# Autodesk Inventor assembly: MotorEncoderAssembly_MIR
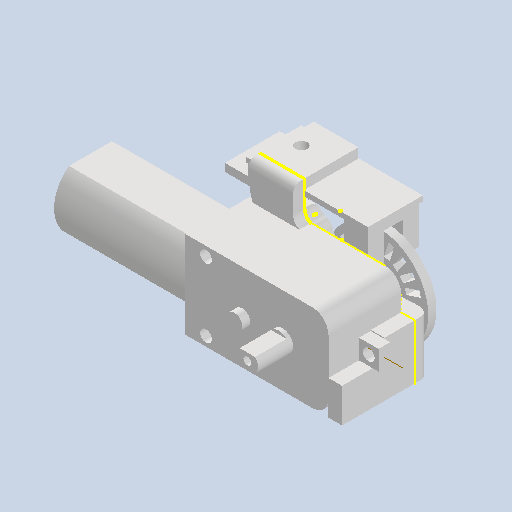
[picture p0: Inventor's stored thumbnail of the model, 512x512]
Saved by Autodesk Inventor 2022 (Build 260153070, 153G)
## iProperties
Created: 2021-11-27
Part Number: MotorEncoderAssembly_MIR
Document SubType Name: Assembly
Designer: a laptop
Author: a laptop
## Documents named in this file (8)
- C:\Users\a laptop\Desktop\SumoBot\sumobotENCODER\MotorEncoderAssembly_MIR.iam
- C:\Users\a laptop\Desktop\SumoBot\sumobotENCODER\REF_PART\LM393 encoder_MIR.ipt
- C:\Users\a laptop\Desktop\SumoBot\sumobotENCODER\REF_PART\TT encoder disk_MIR.ipt
- C:\Users\a laptop\Desktop\SumoBot\sumobotENCODER\REF_PART\TT motor output_MIR.ipt
- C:\Users\a laptop\Desktop\SumoBot\sumobotENCODER\MotorEncoderBracket_MIR.ipt
- C:\Users\a laptop\Desktop\SumoBot\sumobotENCODER\REF_PART\TTencoderspacer_MIR.ipt
- C:\Users\a laptop\Desktop\SumoBot\sumobotENCODER\REF_PART\TTencodercap_MIR.ipt
- C:\Users\a laptop\Desktop\SumoBot\sumobotENCODER\REF_PART\TTmotor_MIR.ipt
## Components (7 placed, 7 different names)
1. LM393 encoder_MIR:1 — Tangent:1, Mate:3, Angle:3, Angle:2, Mate:8
2. TT encoder disk_MIR:1 — Tangent:1, Mate:3, Mate:2, Flush:1, Angle:1, Mate:1
3. TT motor output_MIR:1 — Angle:3, Angle:2, Mate:2, Flush:1, Angle:1, Mate:1, Mate:4, Mate:5, Flush:2, Flush:3, Flush:4, Mate:11, Mate:10
4. MotorEncoderBracket_MIR:1 — Flush:2
5. TTencoderspacer_MIR:1 — Flush:3
6. TTencodercap_MIR:1 — Flush:4
7. TTmotor_MIR:1 — Mate:11, Mate:10
## Relationships (16: Mate 11, Angle 3, Tangent 1, Flush 1)
- Tangent:1 (1.5 mm): LM393 encoder_MIR:1 ↔ TT encoder disk_MIR:1
- Mate:3 (1.5 mm): LM393 encoder_MIR:1 ↔ TT encoder disk_MIR:1
- Angle:3 (180 deg): LM393 encoder_MIR:1 ↔ TT motor output_MIR:1
- Angle:2 (180 deg): LM393 encoder_MIR:1 ↔ TT motor output_MIR:1
- Mate:2: TT encoder disk_MIR:1 ↔ TT motor output_MIR:1
- Flush:1: TT encoder disk_MIR:1 ↔ TT motor output_MIR:1
- Angle:1 (0 deg): TT encoder disk_MIR:1 ↔ TT motor output_MIR:1
- Mate:1: TT encoder disk_MIR:1 ↔ TT motor output_MIR:1
- Mate:4: TT motor output_MIR:1
- Mate:5: TT motor output_MIR:1
- Mate:8: LM393 encoder_MIR:1
- Flush:2 [Mate]: TT motor output_MIR:1 ↔ MotorEncoderBracket_MIR:1
- Flush:3 [Mate]: TT motor output_MIR:1 ↔ TTencoderspacer_MIR:1
- Flush:4 [Mate]: TT motor output_MIR:1 ↔ TTencodercap_MIR:1
- Mate:11: TT motor output_MIR:1 ↔ TTmotor_MIR:1
- Mate:10: TT motor output_MIR:1 ↔ TTmotor_MIR:1
